# Autodesk Inventor assembly: GPS
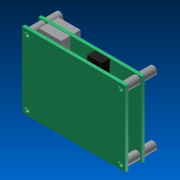
[picture p0: Inventor's stored thumbnail of the model, 180x180]
Saved by Autodesk Inventor 2012 (Build 160160000, 160)
## iProperties
Created: 2015-11-18
Part Number: GPS
Document SubType Name: Assembly
Designer: Alex Becerra
Mass: 13.3653 g
Surface Area: 119.268 cm^2
Volume: 13.3653 cm^3
Density: 1 g/cm^3
Author: Alex Becerra
## Documents named in this file (4)
- C:\Users\Thinkpad\Cubesat SUChAI\Mecanica\Modelo_3D\Placa_payloads\GPS\GPS.iam
- C:\Users\Thinkpad\Cubesat SUChAI\Mecanica\Modelo_3D\Placa_payloads\GPS\adapgps.ipt
- C:\Users\Thinkpad\Cubesat SUChAI\Mecanica\Modelo_3D\Placa_payloads\GPS\gps.ipt
- C:\Users\Thinkpad\Cubesat SUChAI\Mecanica\Modelo_3D\Placa_payloads\GPS\Separador2.ipt
## Components (10 placed, 3 different names)
1. adapgps:1 — Mate:9, Mate:10, Mate:11
2. gps:1 — Mate:1, Mate:2, Mate:3, Mate:4, Mate:5, Mate:6, Mate:7, Mate:8, Mate:12, Mate:13, Mate:14, Mate:15, Mate:16, Mate:17, Mate:18, Mate:19
3. Separador2:1 — Mate:4, Mate:7
4. Separador2:2 — Mate:14, Mate:18
5. Separador2:3 — Mate:1, Mate:2, Mate:9
6. Separador2:4 — Mate:15, Mate:19
7. Separador2:6 — Mate:13, Mate:17
8. Separador2:7 — Mate:12, Mate:16
9. Separador2:8 — Mate:3, Mate:6, Mate:10
10. Separador2:9 — Mate:5, Mate:8, Mate:11
## Relationships (19: Mate 19)
- Mate:1: gps:1 ↔ Separador2:3
- Mate:2: gps:1 ↔ Separador2:3
- Mate:3: gps:1 ↔ Separador2:8
- Mate:4: gps:1 ↔ Separador2:1
- Mate:5: gps:1 ↔ Separador2:9
- Mate:6: gps:1 ↔ Separador2:8
- Mate:7: gps:1 ↔ Separador2:1
- Mate:8: gps:1 ↔ Separador2:9
- Mate:9: adapgps:1 ↔ Separador2:3
- Mate:10: adapgps:1 ↔ Separador2:8
- Mate:11: adapgps:1 ↔ Separador2:9
- Mate:12: gps:1 ↔ Separador2:7
- Mate:13: gps:1 ↔ Separador2:6
- Mate:14: gps:1 ↔ Separador2:2
- Mate:15: gps:1 ↔ Separador2:4
- Mate:16: gps:1 ↔ Separador2:7
- Mate:17: gps:1 ↔ Separador2:6
- Mate:18: gps:1 ↔ Separador2:2
- Mate:19: gps:1 ↔ Separador2:4
